# Autodesk Inventor assembly: test_development_pid
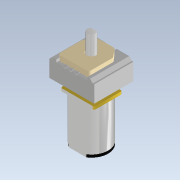
[picture p0: Inventor's stored thumbnail of the model, 180x180]
Saved by Autodesk Inventor 2020.2 (Build 242310000, 310)
## iProperties
Created: 2020-04-25
Part Number: test_development_pid
Document SubType Name: Assembly
Designer: Bardo91
Author: Bardo91
## Documents named in this file (4)
- D:\programming\elric\hardware\0.development\test_development_pid.iam
- D:\programming\elric\hardware\1. hand\motor_dc_6v_30rpm.ipt
- D:\programming\elric\hardware\1. hand\potentiometer_bourns_3382_12mm.ipt
- D:\programming\elric\hardware\0.development\pid_test_structure.ipt
## Components (3 placed, 3 different names)
1. motor_dc_6v_30rpm:1 — Mate:1, Mate:2, Mate:3, Mate:4
2. potentiometer_bourns_3382_12mm:1 — Mate:1, Mate:5
3. pid_test_structure:1 — Mate:2, Mate:3, Mate:4, Mate:5
## Relationships (5: Mate 5)
- Mate:1: motor_dc_6v_30rpm:1 ↔ potentiometer_bourns_3382_12mm:1
- Mate:2: motor_dc_6v_30rpm:1 ↔ pid_test_structure:1
- Mate:3: motor_dc_6v_30rpm:1 ↔ pid_test_structure:1
- Mate:4: motor_dc_6v_30rpm:1 ↔ pid_test_structure:1
- Mate:5: potentiometer_bourns_3382_12mm:1 ↔ pid_test_structure:1
